# Autodesk Inventor assembly: Chasis
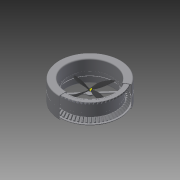
[picture p0: Inventor's stored thumbnail of the model, 180x180]
Saved by Autodesk Inventor 2015 (Build 190159000, 159)
## iProperties
Created: 2016-03-23
Part Number: Chasis
Document SubType Name: Assembly
Designer: david_000
Author: david_000
## Documents named in this file (6)
- C:\Users\david_000\Documents\Drone-Git\Drone\3D Models\Project\Chasis\Chasis.iam
- C:\Users\david_000\Documents\Drone-Git\Drone\3D Models\Project\Chasis\Top.ipt
- C:\Users\david_000\Documents\Drone-Git\Drone\3D Models\Project\Chasis\Bottom.ipt
- C:\Users\david_000\Documents\Drone-Git\Drone\3D Models\Project\Chasis\Top_Bevel.iam
- C:\Users\david_000\Documents\Drone-Git\Drone\3D Models\Project\Beveled_Ring.ipt
- C:\Users\david_000\Documents\Drone-Git\Drone\3D Models\Project\Prop.iam
## Components (5 placed, 5 different names)
1. Top:1 — Insert:1, Flush:1, Insert:2, Insert:4
2. Bottom:1 — Insert:1, Flush:1
3. Top_Bevel:1 [sub-assembly] — Insert:2, Insert:3
4. Beveled_Ring:1 — Insert:3
5. Prop:1 [sub-assembly] — Insert:4
## Relationships (5: Insert 4, Flush 1)
- Insert:1: Top:1 ↔ Bottom:1
- Flush:1: Top:1 ↔ Bottom:1
- Insert:2 (3.175 mm): Top:1 ↔ Top_Bevel:1
- Insert:3 (3.175 mm): Top_Bevel:1 ↔ Beveled_Ring:1
- Insert:4 (50.8 mm): Top:1 ↔ Prop:1
